# Autodesk Inventor assembly: BuchsenLeiste16
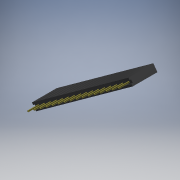
[picture p0: Inventor's stored thumbnail of the model, 180x180]
Saved by Autodesk Inventor 2017 (Build 210142000, 142)
## iProperties
Part Number: BuchsenLeiste16
Material: Generisch
Document SubType Name: Assembly
Designer: Enno
Author: Enno
## Documents named in this file (2)
- C:\Users\Enno\Desktop\IMU_Motion_Classification\Adafruit_Feather\CAD\stiftleiste_male-1.snapshot.20\Weib\Gerade\BuchsenLeiste16.iam
- C:\Users\Enno\Desktop\IMU_Motion_Classification\Adafruit_Feather\CAD\stiftleiste_male-1.snapshot.20\Weib\Gerade\Buchsenleiste_female.ipt
## Components (16 placed, 1 different names)
1. Buchsenleiste_female:1 — Passend:3, Passend:4, Fluchtend:2
2. Buchsenleiste_female:2 — Passend:1, Passend:2, Fluchtend:1, Fluchtend:3, Passend:5, Passend:6
3. Buchsenleiste_female:3 — Passend:3, Passend:4, Fluchtend:2, Fluchtend:3, Passend:5, Passend:6
4. Buchsenleiste_female:4 — Passend:1, Passend:2, Fluchtend:1, Passend:7, Passend:8, Fluchtend:4
5. Buchsenleiste_female:5 — Passend:7, Passend:8, Fluchtend:4, Passend:9, Passend:10, Passend:11
6. Buchsenleiste_female:6 — Passend:9, Passend:10, Passend:11, Passend:12, Passend:13, Passend:14
7. Buchsenleiste_female:7 — Passend:15, Passend:16, Passend:17, Passend:18, Passend:19, Passend:20
8. Buchsenleiste_female:8 — Passend:12, Passend:13, Passend:14, Passend:15, Passend:16, Passend:17
9. Buchsenleiste_female:9 — Passend:30, Passend:31, Passend:32, Passend:33, Passend:34, Passend:35
10. Buchsenleiste_female:10 — Passend:24, Passend:25, Passend:26, Passend:27, Passend:28, Passend:29
11. Buchsenleiste_female:11 — Passend:27, Passend:28, Passend:29, Passend:30, Passend:31, Passend:32
12. Buchsenleiste_female:12 — Passend:18, Passend:19, Passend:20, Passend:21, Passend:22, Passend:23
13. Buchsenleiste_female:13 — Passend:21, Passend:22, Passend:23, Passend:24, Passend:25, Passend:26
14. Buchsenleiste_female:14 — Passend:33, Passend:34, Passend:35, Passend:36, Passend:37, Passend:38
15. Buchsenleiste_female:15 — Passend:36, Passend:37, Passend:38, Passend:39, Passend:40, Passend:41
16. Buchsenleiste_female:16 — Passend:39, Passend:40, Passend:41
## Relationships (45: Mate 41, Flush 4)
- Passend:1 [Mate]: Buchsenleiste_female:2 ↔ Buchsenleiste_female:4
- Passend:2 [Mate]: Buchsenleiste_female:2 ↔ Buchsenleiste_female:4
- Fluchtend:1 [Flush]: Buchsenleiste_female:2 ↔ Buchsenleiste_female:4
- Passend:3 [Mate]: Buchsenleiste_female:1 ↔ Buchsenleiste_female:3
- Passend:4 [Mate]: Buchsenleiste_female:1 ↔ Buchsenleiste_female:3
- Fluchtend:2 [Flush]: Buchsenleiste_female:1 ↔ Buchsenleiste_female:3
- Fluchtend:3 [Flush]: Buchsenleiste_female:2 ↔ Buchsenleiste_female:3
- Passend:5 [Mate]: Buchsenleiste_female:2 ↔ Buchsenleiste_female:3
- Passend:6 [Mate]: Buchsenleiste_female:2 ↔ Buchsenleiste_female:3
- Passend:7 [Mate]: Buchsenleiste_female:4 ↔ Buchsenleiste_female:5
- Passend:8 [Mate]: Buchsenleiste_female:4 ↔ Buchsenleiste_female:5
- Fluchtend:4 [Flush]: Buchsenleiste_female:4 ↔ Buchsenleiste_female:5
- Passend:9 [Mate]: Buchsenleiste_female:5 ↔ Buchsenleiste_female:6
- Passend:10 [Mate]: Buchsenleiste_female:5 ↔ Buchsenleiste_female:6
- Passend:11 [Mate]: Buchsenleiste_female:5 ↔ Buchsenleiste_female:6
- Passend:12 [Mate]: Buchsenleiste_female:6 ↔ Buchsenleiste_female:8
- Passend:13 [Mate]: Buchsenleiste_female:6 ↔ Buchsenleiste_female:8
- Passend:14 [Mate]: Buchsenleiste_female:6 ↔ Buchsenleiste_female:8
- Passend:15 [Mate]: Buchsenleiste_female:7 ↔ Buchsenleiste_female:8
- Passend:16 [Mate]: Buchsenleiste_female:7 ↔ Buchsenleiste_female:8
- Passend:17 [Mate]: Buchsenleiste_female:7 ↔ Buchsenleiste_female:8
- Passend:18 [Mate]: Buchsenleiste_female:7 ↔ Buchsenleiste_female:12
- Passend:19 [Mate]: Buchsenleiste_female:7 ↔ Buchsenleiste_female:12
- Passend:20 [Mate]: Buchsenleiste_female:7 ↔ Buchsenleiste_female:12
- Passend:21 [Mate]: Buchsenleiste_female:12 ↔ Buchsenleiste_female:13
- Passend:22 [Mate]: Buchsenleiste_female:12 ↔ Buchsenleiste_female:13
- Passend:23 [Mate]: Buchsenleiste_female:12 ↔ Buchsenleiste_female:13
- Passend:24 [Mate]: Buchsenleiste_female:10 ↔ Buchsenleiste_female:13
- Passend:25 [Mate]: Buchsenleiste_female:10 ↔ Buchsenleiste_female:13
- Passend:26 [Mate]: Buchsenleiste_female:10 ↔ Buchsenleiste_female:13
- Passend:27 [Mate]: Buchsenleiste_female:10 ↔ Buchsenleiste_female:11
- Passend:28 [Mate]: Buchsenleiste_female:10 ↔ Buchsenleiste_female:11
- Passend:29 [Mate]: Buchsenleiste_female:10 ↔ Buchsenleiste_female:11
- Passend:30 [Mate]: Buchsenleiste_female:9 ↔ Buchsenleiste_female:11
- Passend:31 [Mate]: Buchsenleiste_female:9 ↔ Buchsenleiste_female:11
- Passend:32 [Mate]: Buchsenleiste_female:9 ↔ Buchsenleiste_female:11
- Passend:33 [Mate]: Buchsenleiste_female:9 ↔ Buchsenleiste_female:14
- Passend:34 [Mate]: Buchsenleiste_female:9 ↔ Buchsenleiste_female:14
- Passend:35 [Mate]: Buchsenleiste_female:9 ↔ Buchsenleiste_female:14
- Passend:36 [Mate]: Buchsenleiste_female:14 ↔ Buchsenleiste_female:15
- Passend:37 [Mate]: Buchsenleiste_female:14 ↔ Buchsenleiste_female:15
- Passend:38 [Mate]: Buchsenleiste_female:14 ↔ Buchsenleiste_female:15
- Passend:39 [Mate]: Buchsenleiste_female:15 ↔ Buchsenleiste_female:16
- Passend:40 [Mate]: Buchsenleiste_female:15 ↔ Buchsenleiste_female:16
- Passend:41 [Mate]: Buchsenleiste_female:15 ↔ Buchsenleiste_female:16
